# Autodesk Inventor assembly: Assembly
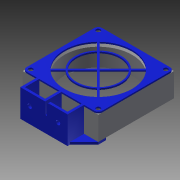
[picture p0: Inventor's stored thumbnail of the model, 180x180]
Saved by Autodesk Inventor 2015 (Build 190159000, 159)
## iProperties
Created: 2014-08-15
Part Number: Assembly
Document SubType Name: Assembly
Designer: Christo
Author: Christo
## Documents named in this file (4)
- D:\Projects\desk_winder\cad\Assembly.iam
- D:\Projects\desk_winder\cad\fan.ipt
- D:\Projects\desk_winder\cad\grid.ipt
- D:\Projects\desk_winder\cad\support.ipt
## Components (3 placed, 3 different names)
1. fan:1 — Flush:1, Flush:2
2. grid:1 — Flush:1
3. support:1 — Flush:2
## Relationships (2: Flush 2)
- Flush:1: fan:1 ↔ grid:1
- Flush:2: fan:1 ↔ support:1
